# Autodesk Inventor assembly: akkufach
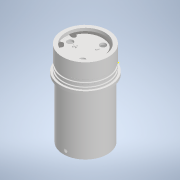
[picture p0: Inventor's stored thumbnail of the model, 180x180]
Saved by Autodesk Inventor 2020.2 (Build 242310000, 310)
## iProperties
Created: 2020-11-11
Part Number: akkufach
Document SubType Name: Assembly
Designer: g.schardt
Author: g.schardt
## Documents named in this file (5)
- C:\Users\g.schardt\Inventor\Tauchlampe\akkufach.iam
- C:\Users\g.schardt\Inventor\Tauchlampe\akkufach_lampe_neu.ipt
- C:\Users\g.schardt\Inventor\Tauchlampe\battery\battery18650User Library-18650-1Cell only.ipt
- C:\Users\g.schardt\Inventor\Tauchlampe\akkufach_deckel.ipt
- C:\Users\g.schardt\Documents\Inventor\Content Center Files\R2020\de-DE\DIN 472(2)\DIN 472 - 40x1,75.ipt
## Components (6 placed, 4 different names)
1. akkufach_lampe_neu:1 — Passend:1, Fluchtend:1, Fluchtend:2, Passend:2, Fluchtend:3, Einfügen:1
2. akkufach_deckel:1 — Passend:2, Fluchtend:3
3. DIN 472 40x1,75:1 — Einfügen:1
4. battery18650User Library-18650-1Cell only:1 — Tangential:1, Fluchtend:2
5. battery18650User Library-18650-1Cell only:2
6. battery18650User Library-18650-1Cell only:3
## Component patterns: (3 elements, first: battery18650User Library-18650-1Cell only:1)
## Relationships (7: Flush 3, Mate 2, Tangent 1, Insert 1)
- Passend:1 [Mate]: akkufach_lampe_neu:1
- Fluchtend:1 [Flush] (-45 mm): akkufach_lampe_neu:1
- Tangential:1 (1.5 mm): battery18650User Library-18650-1Cell only:1
- Fluchtend:2 [Flush] (10 mm): akkufach_lampe_neu:1 ↔ battery18650User Library-18650-1Cell only:1
- Passend:2 [Mate]: akkufach_lampe_neu:1 ↔ akkufach_deckel:1
- Fluchtend:3 [Flush]: akkufach_lampe_neu:1 ↔ akkufach_deckel:1
- Einfügen:1 [Insert]: akkufach_lampe_neu:1 ↔ DIN 472 40x1,75:1
